# Autodesk Inventor assembly: WingGear
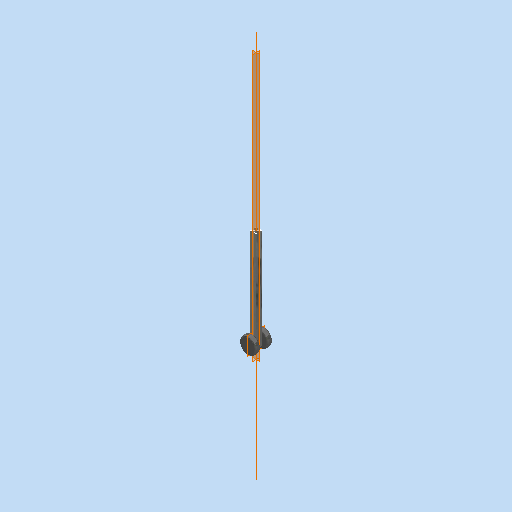
[picture p0: Inventor's stored thumbnail of the model, 512x512]
Saved by Autodesk Inventor 2026.1 (Build 301233000, 233)
## iProperties
Created: 2026-03-27
Part Number: WingGear
Document SubType Name: Assembly
Designer: mateo
Author: mateo
## Documents named in this file (3)
- C:\GitHub\Senior-Design-UAV\Elytra CAD\Parts\Landing Gear\V2\WingGear.iam
- C:\GitHub\Senior-Design-UAV\Elytra CAD\20x20 Extrusions\20x20x260ExtrudedAluminum.ipt
- C:\GitHub\Senior-Design-UAV\Elytra CAD\Parts\Landing Gear\V2\wheel.ipt
## Components (3 placed, 2 different names)
1. 20x20x260ExtrudedAluminum:1 — Mate:1, Mate:2, Mate:3, Mate:4
2. wheel:1 — Mate:1, Mate:3
3. wheel:2 — Mate:2, Mate:4
## Relationships (4: Mate 4)
- Mate:1: 20x20x260ExtrudedAluminum:1 ↔ wheel:1
- Mate:2: 20x20x260ExtrudedAluminum:1 ↔ wheel:2
- Mate:3 (12 mm): 20x20x260ExtrudedAluminum:1 ↔ wheel:1
- Mate:4 (-28 mm): 20x20x260ExtrudedAluminum:1 ↔ wheel:2
